# Autodesk Inventor assembly: Robot_Klara
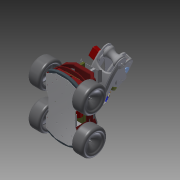
[picture p0: Inventor's stored thumbnail of the model, 180x180]
Saved by Autodesk Inventor 2015 (Build 190159000, 159)
## iProperties
Created: 2015-01-01
Part Number: Robot_Klara
Document SubType Name: Assembly
Designer: Turboslimak
Author: Turboslimak
## Documents named in this file (75)
- C:\Users\Turboslimak\Documents\Inventor\Robot_Klara\Robot_Klara.iam
- C:\Users\Turboslimak\Documents\Inventor\Robot_Klara\podvozek.ipt
- C:\Users\Turboslimak\Documents\Inventor\Robot_Klara\bocnice_kratsi.ipt
- C:\Users\Turboslimak\Documents\Inventor\Robot_Klara\kratka_prepazka.ipt
- C:\Users\Turboslimak\Documents\Inventor\Robot_Klara\predni_komatex.ipt
- C:\Users\Turboslimak\Documents\Inventor\Robot_Klara\bocnice_delsi.ipt
- C:\Users\Turboslimak\Documents\Inventor\Robot_Klara\prepazka_2x_lozisko_2x_dira.ipt
- C:\Users\Turboslimak\Documents\Inventor\Robot_Klara\hridel_kolo.ipt
- C:\Users\Turboslimak\Documents\Inventor\Robot_Klara\Lozisko_15mm.ipt
- C:\Users\Turboslimak\Documents\Inventor\Robot_Klara\hlavni_hridel.ipt
- C:\Users\Turboslimak\Documents\Inventor\Robot_Klara\prepazka_2x_lozisko_2x_dira_predni.ipt
- C:\Users\Turboslimak\Documents\Inventor\Robot_Klara\prepazka_2x_lozisko_1x_dira.ipt
- C:\Users\Turboslimak\Documents\Inventor\Robot_Klara\drzak_motory.ipt
- C:\Users\Turboslimak\Documents\Inventor\Robot_Klara\DC_motor+enkoder.ipt
- C:\Users\Turboslimak\Documents\Inventor\Robot_Klara\gear hridel.ipt
- C:\Users\Turboslimak\Documents\Inventor\Robot_Klara\gear motor.ipt
- C:\Users\Turboslimak\Documents\Inventor\Robot_Klara\Robot_Klara\Design Accelerator\Spur Gears2.iam
- C:\Users\Turboslimak\Documents\Inventor\Robot_Klara\Robot_Klara\Design Accelerator\Spur Gears3.iam
- C:\Users\Turboslimak\Documents\Inventor\Robot_Klara\vymezovaci_trubicka.ipt
- C:\Users\Turboslimak\Documents\Inventor\Robot_Klara\hridel kuzelova kolecka.ipt
- C:\Users\Turboslimak\Documents\Inventor\Robot_Klara\Robot_Klara\Design Accelerator\Bevel Gears2.iam
- C:\Users\Turboslimak\Documents\Inventor\Robot_Klara\Robot_Klara\Design Accelerator\Bevel Gears3.iam
- C:\Users\Turboslimak\Documents\Inventor\Robot_Klara\Robot_Klara\Design Accelerator\Bevel Gears4.iam
- C:\Users\Turboslimak\Documents\Inventor\Robot_Klara\Robot_Klara\Design Accelerator\Bevel Gears7.iam
- C:\Users\Turboslimak\Documents\Inventor\Robot_Klara\naraznik_kryt.ipt
- C:\Users\Turboslimak\Documents\Inventor\Robot_Klara\naraznik.ipt
- C:\Users\Turboslimak\Documents\Inventor\Robot_Klara\kolo.ipt
- C:\Users\Turboslimak\Documents\Inventor\Robot_Klara\izolovaci_deska.ipt
- C:\Users\Turboslimak\Documents\Inventor\Robot_Klara\vrch.ipt
- C:\Users\Turboslimak\Documents\Inventor\Robot_Klara\drzak_svetlomet0.ipt
- C:\Users\Turboslimak\Documents\Inventor\Robot_Klara\svetlo_trubicka.ipt
- C:\Users\Turboslimak\Documents\Inventor\Robot_Klara\svetlo_mlecne_plexi.ipt
- C:\Users\Turboslimak\Documents\Inventor\Robot_Klara\komatex_senzor.ipt
- C:\Users\Turboslimak\Documents\Inventor\Robot_Klara\podpera_rameno.ipt
- C:\Users\Turboslimak\Documents\Inventor\Robot_Klara\podpera_deska_rameno.ipt
- C:\Users\Turboslimak\Documents\Inventor\Robot_Klara\deska-pod_otocny kruh.ipt
- C:\Users\Turboslimak\Documents\Inventor\Robot_Klara\podvozek_priklopny_kryt.ipt
- C:\Users\Turboslimak\Documents\Inventor\Robot_Klara\valecky_na_otocny_kruh.ipt
- C:\Users\Turboslimak\Documents\Inventor\Robot_Klara\otocni_kruh(svrchni).ipt
- C:\Users\Turboslimak\Documents\Inventor\Robot_Klara\hridelka1.ipt
- C:\Users\Turboslimak\Documents\Inventor\Robot_Klara\standart_servo.ipt
- C:\Users\Turboslimak\Documents\Inventor\Robot_Klara\servo_paka_dolu.ipt
- C:\Users\Turboslimak\Documents\Inventor\Robot_Klara\stojan2.ipt
- C:\Users\Turboslimak\Documents\Inventor\Robot_Klara\stojan2a.ipt
- C:\Users\Turboslimak\Documents\Inventor\Robot_Klara\servodrzak.ipt
- C:\Users\Turboslimak\Documents\Inventor\Robot_Klara\micro_servo.ipt
- C:\Users\Turboslimak\Documents\Inventor\Robot_Klara\rameno(b)dole.ipt
- C:\Users\Turboslimak\Documents\Inventor\Robot_Klara\rameno(a)dole.ipt
- C:\Users\Turboslimak\Documents\Inventor\Robot_Klara\vystuha_hridel_nahore.ipt
- C:\Users\Turboslimak\Documents\Inventor\Robot_Klara\rameno(a)nahore.ipt
- C:\Users\Turboslimak\Documents\Inventor\Robot_Klara\rameno(b)nahore.ipt
- C:\Users\Turboslimak\Documents\Inventor\Robot_Klara\kolecko_servo(2).ipt
- C:\Users\Turboslimak\Documents\Inventor\Robot_Klara\kolecko_rameno(2).ipt
- C:\Users\Turboslimak\Documents\Inventor\Robot_Klara\clanek3a.ipt
- C:\Users\Turboslimak\Documents\Inventor\Robot_Klara\packa_strana(a).ipt
- C:\Users\Turboslimak\Documents\Inventor\Robot_Klara\otaceni_packy_microservo.ipt
- C:\Users\Turboslimak\Documents\Inventor\Robot_Klara\kolecko_rameno(3).ipt
- C:\Users\Turboslimak\Documents\Inventor\Robot_Klara\kolecko_servo(3).ipt
- C:\Users\Turboslimak\Documents\Inventor\Robot_Klara\hridel1.ipt
- C:\Users\Turboslimak\Documents\Inventor\Robot_Klara\hridel2.ipt
- C:\Users\Turboslimak\Documents\Inventor\Robot_Klara\hridelka_packa.ipt
- C:\Users\Turboslimak\Documents\Inventor\Robot_Klara\ruka_zak, deska.ipt
- C:\Users\Turboslimak\Documents\Inventor\Robot_Klara\tahlo3.ipt
- C:\Users\Turboslimak\Documents\Inventor\Robot_Klara\tahlo6.ipt
- C:\Users\Turboslimak\Documents\Inventor\Robot_Klara\tahlo7.ipt
- C:\Users\Turboslimak\Documents\Inventor\Robot_Klara\tahlo-neco.ipt
- C:\Users\Turboslimak\Documents\Inventor\Robot_Klara\tahlo5.ipt
- C:\Users\Turboslimak\Documents\Inventor\Robot_Klara\ruka_lozisko.ipt
- C:\Users\Turboslimak\Documents\Inventor\Robot_Klara\kolejnicka_ruka.ipt
- C:\Users\Turboslimak\Documents\Inventor\Robot_Klara\kolejnicka_ruka_druha_cast.ipt
- C:\Users\Turboslimak\Documents\Inventor\Robot_Klara\paka2_micro.ipt
- C:\Users\Turboslimak\Documents\Inventor\Robot_Klara\pracka_leva1.ipt
- C:\Users\Turboslimak\Documents\Inventor\Robot_Klara\packa_prava.ipt
- C:\Users\Turboslimak\Documents\Inventor\Robot_Klara\ruka_tahlo.ipt
- C:\Users\Turboslimak\Documents\Inventor\Robot_Klara\paka_packa.ipt
## Components (133 placed, 70 different names)
1. podvozek:1 — Mate:1, Mate:2, Mate:3, Mate:4, Mate:5, Mate:6, Mate:18, Mate:19, Mate:20, Mate:21, Mate:22, Mate:23, Mate:33, Mate:34, Mate:35, Mate:36, Mate:40, Mate:42, Mate:50, Flush:1, Mate:69, Mate:79, Mate:80, Mate:81, Mate:82, Mate:83, Mate:84, Mate:85, Mate:86, Mate:99, Mate:100, Mate:101, Mate:105, Mate:112, Mate:113, Mate:114, Mate:115, Mate:177, Mate:178, Mate:179, Mate:180, Mate:187, Mate:188, Mate:189, Mate:191, Mate:192, Mate:193, Mate:203, Mate:204, Mate:205
2. bocnice_kratsi:1 — Mate:4, Mate:5, Mate:6, Mate:24, Mate:74, Mate:75, Mate:225
3. bocnice_kratsi:2 — Mate:1, Mate:2, Mate:3, Mate:46, Mate:65, Mate:76, Mate:223
4. bocnice_delsi:1 — Mate:18, Mate:19, Mate:20, Mate:21, Mate:51, Mate:58, Mate:73
5. predni_komatex:1 — Mate:22, Mate:23, Mate:24, Mate:87, Mate:88, Mate:212, Mate:213, Mate:214, Mate:215, Mate:216, Mate:217
6. bocnice_delsi:2 — Mate:33, Mate:34, Mate:35, Mate:36, Mate:59, Mate:67
7. prepazka_2x_lozisko_2x_dira:1 — Mate:40, Mate:42, Mate:56, Mate:57, Mate:69, Mate:70, Mate:71, Mate:72, Mate:89, Mate:90, Flush:2, Flush:3
8. hridel_kolo:2 — Mate:51, Mate:139, Mate:146, Flush:9, Mate:164
9. hridel_kolo:4 — Mate:46, Mate:138, Mate:150, Flush:4
10. Lozisko_15mm:1 — Mate:57, Mate:102
11. Lozisko_15mm:2 — Mate:70, Mate:71, Mate:78
12. Lozisko_15mm:4 — Mate:222
13. Lozisko_15mm:5 — Mate:56, Mate:72, Mate:77
14. Lozisko_15mm:6 — Mate:58, Mate:73, Mate:142
15. Lozisko_15mm:8 — Mate:65, Mate:76, Mate:143
16. Lozisko_15mm:10 — Mate:59, Mate:67, Mate:145
17. kratka_prepazka:1 — Mate:79, Mate:80, Mate:90, Mate:91, Mate:92, Mate:129
18. kratka_prepazka:2 — Mate:82, Mate:84, Mate:89, Mate:93, Mate:94
19. kratka_prepazka:3 — Mate:83, Mate:85, Mate:88, Mate:95, Mate:98
20. kratka_prepazka:4 — Mate:81, Mate:86, Mate:87, Mate:96, Mate:97, Mate:239
21. hlavni_hridel:1 — Mate:78, Mate:111, Flush:3, Mate:123, Mate:152, Flush:6, Mate:154, Mate:160, Mate:167
22. hlavni_hridel:2 — Mate:77, Mate:103, Mate:110, Flush:2, Mate:122, Mate:147, Mate:153, Flush:5, Mate:157, Mate:163
23. Lozisko_15mm:11 — Mate:93, Mate:94
24. Lozisko_15mm:12 — Mate:91, Mate:92, Mate:175
25. Lozisko_15mm:13 — Mate:95, Mate:98
26. Lozisko_15mm:14 — Mate:74, Mate:75, Mate:144
27. Lozisko_15mm:15 — Mate:96, Mate:97, Mate:173
28. prepazka_2x_lozisko_2x_dira_predni:1 — Mate:99, Mate:100, Mate:101, Mate:102, Mate:104
29. Lozisko_15mm:16 — Mate:106, Mate:109, Mate:111
30. Lozisko_15mm:17 — Mate:107, Mate:108, Mate:110
31. Lozisko_15mm:18 — Mate:103, Mate:104
32. prepazka_2x_lozisko_1x_dira:1 — Mate:105, Mate:106, Mate:107, Mate:108, Mate:109, Mate:112, Mate:126, Mate:127, Mate:128, Mate:224
33. drzak_motory:1 — Mate:113, Mate:114, Mate:115, Mate:116, Mate:117, Mate:118, Mate:119, Mate:120, Mate:121
34. DC_motor+enkoder:1 — Mate:117, Mate:119, Mate:120, Mate:125
35. DC_motor+enkoder:2 — Mate:116, Mate:118, Mate:121, Mate:124
36. gear hridel:1 — Mate:122, Mate:126, Mate:132, Mate:133
37. gear hridel:2 — Mate:123, Mate:127, Mate:136, Mate:137
38. gear motor:1 — Mate:125, Mate:129, Mate:134, Mate:135
39. gear motor:2 — Mate:124, Mate:128, Mate:130, Mate:131
40. Spur Gears:1 [sub-assembly] — Mate:130, Mate:131, Mate:132, Mate:133
41. Spur Gears:2 [sub-assembly] — Mate:134, Mate:135, Mate:136, Mate:137
42. vymezovaci_trubicka:1 — Mate:138, Mate:143, Mate:195, Mate:196
43. vymezovaci_trubicka:2 — Mate:139, Mate:142, Mate:197, Mate:198
44. vymezovaci_trubicka:3 — Mate:144, Mate:172, Mate:201, Mate:202
45. vymezovaci_trubicka:4 — Mate:145, Mate:176, Mate:199
46. hridel kuzelova kolecka:1 — Mate:150, Flush:4, Mate:157, Mate:162, Angle:3
47. hridel kuzelova kolecka:2 — Mate:154, Angle:1, Mate:159, Flush:10
48. hridel kuzelova kolecka:3 — Mate:152, Flush:6, Mate:158
49. hridel kuzelova kolecka:4 — Mate:153, Flush:5, Mate:161, Angle:2
50. hridel kuzelova kolecka:5 — Mate:167, Mate:169, Mate:170
51. hridel kuzelova kolecka:6 — Mate:168, Angle:4, Mate:171, Flush:11, Mate:221
52. hridel kuzelova kolecka:7 — Mate:146, Flush:9, Mate:165
53. hridel kuzelova kolecka:8 — Mate:147, Mate:166
54. Bevel Gears:1 [sub-assembly] — Angle:1, Mate:158, Mate:159, Mate:160, Mate:174
55. Bevel Gears:2 [sub-assembly] — Mate:161, Angle:2, Mate:162, Angle:3
56. Bevel Gears:3 [sub-assembly] — Mate:163, Mate:164, Mate:165, Mate:166
57. Bevel Gears:4 [sub-assembly] — Mate:168, Angle:4, Mate:169, Mate:170, Mate:171
58. hridel_kolo:5 — Flush:11, Mate:175, Mate:176, Mate:200, Mate:221, Mate:222
59. hridel_kolo:6 — Flush:10, Mate:172, Mate:173, Mate:174
60. naraznik_kryt:1 — Mate:177, Mate:178, Mate:190
61. naraznik_kryt:2 — Mate:179, Mate:180, Mate:194
62. naraznik:2 — Mate:187, Mate:188, Mate:189, Mate:190
63. naraznik:3 — Mate:191, Mate:192, Mate:193, Mate:194
64. kolo:1 — Mate:199, Mate:200
65. kolo:2 — Mate:197, Mate:198
66. kolo:3 — Mate:201, Mate:202
67. kolo:4 — Mate:195, Mate:196
68. izolovaci_deska:1 — Mate:203, Mate:204, Mate:205
69. vrch:1 — Mate:223, Mate:224, Mate:225, Mate:226, Flush:12, Mate:228, Mate:229, Mate:230, Mate:231, Mate:236, Mate:237, Mate:238, Mate:241, Mate:242, Mate:243, Mate:244
70. drzak_svetlomet0:1 — Mate:212, Mate:213, Mate:214, Mate:215, Mate:216, Mate:218
71. svetlo_trubicka:1 — Mate:217, Mate:218, Mate:219, Mate:220
72. svetlo_mlecne_plexi:1 — Mate:219, Mate:220
73. komatex_senzor:1 — Mate:226, Flush:12
74. podpera_rameno:1 — Mate:228, Mate:229, Mate:235
75. podpera_rameno:2 — Mate:230, Mate:231, Mate:232, Mate:234
76. podpera_deska_rameno:1 — Mate:232, Mate:234, Mate:235
77. deska-pod_otocny kruh:1 — Mate:236, Mate:237, Mate:238
78. podvozek_priklopny_kryt:1 — Mate:239, Mate:241
79. deska-pod_otocny kruh:2 — Mate:242, Mate:243, Mate:244, Mate:245, Mate:246, Mate:247, Mate:248, Mate:249, Mate:250, Mate:251
80. valecky_na_otocny_kruh:1 — Mate:245, Mate:246, Tangent:1
81. valecky_na_otocny_kruh:2 — Mate:249, Mate:250, Tangent:2
82. valecky_na_otocny_kruh:3 — Mate:247, Mate:248
83. otocni_kruh(svrchni):1 — Tangent:1, Tangent:2, Mate:252, Mate:253, Mate:254, Mate:255, Mate:264, Mate:265, Mate:266, Mate:267, Mate:268, Mate:269, Mate:274
84. hridelka1:1 — Mate:251, Mate:252
85. standart_servo:1 — Mate:253, Mate:254, Mate:255, Mate:262, Mate:263
86. servo_paka_dolu:1 — Mate:262, Mate:263, Mate:275, Mate:276, Mate:277
87. stojan2:1 — Mate:264, Mate:265, Mate:270, Mate:274, Mate:282, Mate:318
88. stojan2a:1 — Mate:266, Mate:267, Mate:268
89. servodrzak:1 — Mate:269, Mate:270, Mate:271, Mate:272, Mate:273
90. micro_servo:1 — Mate:271, Mate:272, Mate:273
91. rameno(b)dole:1 — Mate:275, Mate:276, Mate:277, Mate:278, Mate:279, Mate:280, Mate:281, Mate:283, Mate:295
92. standart_servo:2 — Mate:278, Mate:279, Mate:280, Mate:290, Mate:291
93. rameno(a)dole:1 — Mate:281, Mate:282, Mate:283, Mate:289, Mate:316
94. vystuha_hridel_nahore:1 — Mate:284, Mate:285, Mate:286, Mate:287, Mate:289
95. rameno(a)nahore:1 — Mate:284, Mate:285, Mate:288, Mate:308, Mate:309, Mate:310, Mate:313, Mate:317
96. rameno(b)nahore:1 — Mate:286, Mate:287, Mate:288, Mate:292, Mate:293, Mate:294, Mate:312
97. kolecko_servo(2):1 — Mate:290, Mate:291
98. kolecko_rameno(2):1 — Mate:292, Mate:293, Mate:294, Mate:295
99. standart_servo:3 — Mate:296, Mate:297, Mate:298, Mate:306, Mate:307
100. clanek3a:1 — Mate:299, Mate:300, Mate:301, Mate:304, Mate:305, Mate:311, Mate:312, Mate:380
101. packa_strana(a):1 — Mate:296, Mate:297, Mate:298, Mate:304, Mate:305, Mate:311
102. micro_servo:2 — Mate:299, Mate:300, Mate:301, Mate:302, Mate:303
103. otaceni_packy_microservo:1 — Mate:302, Mate:303, Mate:314, Mate:315
104. kolecko_rameno(3):1 — Mate:308, Mate:309, Mate:310
105. kolecko_servo(3):1 — Mate:306, Mate:307, Mate:313
106. hridel1:1 — Mate:316
107. hridel2:1 — Mate:317
108. hridelka_packa:1 — Mate:314, Mate:315, Mate:373
109. hridel1:2 — Mate:318
110. ruka_zak, deska:1 — Mate:319, Mate:320, Mate:326, Mate:328, Mate:330, Mate:331, Mate:332, Mate:333, Mate:334, Mate:336, Mate:343, Mate:344, Mate:346, Mate:347, Mate:349, Mate:350, Mate:351, Mate:352, Mate:353, Mate:354, Mate:362, Mate:363, Mate:364, Mate:366, Mate:377, Mate:378, Mate:392, Mate:393, Mate:394
111. tahlo3:1 — Mate:319, Mate:320, Mate:368, Mate:395
112. tahlo7:1 — Mate:366, Mate:370, Mate:372
113. tahlo-neco:1 — Mate:368, Mate:369, Mate:370, Mate:388
114. ruka_lozisko:1 — Mate:362, Mate:363, Mate:364, Mate:373, Mate:380
115. kolejnicka_ruka:1 — Mate:349, Mate:350, Mate:351, Mate:357, Mate:358
116. kolejnicka_ruka_druha_cast:1 — Mate:357, Mate:358, Mate:384, Mate:385, Mate:386
117. paka2_micro:1 — Mate:355, Mate:356, Mate:374, Mate:389
118. pracka_leva1:1 — Mate:327, Mate:329, Mate:335, Mate:348, Mate:395
119. ruka_tahlo:1 — Mate:326, Mate:327, Mate:328, Mate:329
120. ruka_tahlo:2 — Mate:332, Mate:336, Mate:337
121. ruka_tahlo:3 — Mate:333, Mate:334, Mate:335
122. ruka_tahlo:4 — Mate:330, Mate:331, Mate:337, Mate:383
123. tahlo3:2 — Mate:343, Mate:344, Mate:375, Mate:376
124. tahlo3:3 — Mate:346, Mate:347, Mate:348, Mate:369
125. tahlo3:4 — Mate:377, Mate:378, Mate:379, Mate:381, Mate:382
126. micro_servo:3 — Mate:352, Mate:353, Mate:354, Mate:355, Mate:356
127. tahlo-neco:2
128. tahlo-neco:3 — Mate:372, Mate:375, Mate:376, Mate:379, Mate:387
129. tahlo5:1 — Mate:374
130. packa_prava:1 — Mate:381, Mate:382, Mate:383
131. tahlo6:1 — Mate:384, Mate:385, Mate:386, Mate:387, Mate:388, Mate:390, Mate:391
132. tahlo5:2 — Mate:389, Mate:390, Mate:391
133. paka_packa:1 — Mate:392, Mate:393, Mate:394
## Relationships (326: Mate 310, Flush 10, Angle 4, Tangent 2)
- Mate:1: podvozek:1 ↔ bocnice_kratsi:2
- Mate:2: podvozek:1 ↔ bocnice_kratsi:2
- Mate:3: podvozek:1 ↔ bocnice_kratsi:2
- Mate:4: podvozek:1 ↔ bocnice_kratsi:1
- Mate:5: podvozek:1 ↔ bocnice_kratsi:1
- Mate:6: podvozek:1 ↔ bocnice_kratsi:1
- Mate:18: podvozek:1 ↔ bocnice_delsi:1
- Mate:19: podvozek:1 ↔ bocnice_delsi:1
- Mate:20: podvozek:1 ↔ bocnice_delsi:1
- Mate:21: podvozek:1 ↔ bocnice_delsi:1
- Mate:22: podvozek:1 ↔ predni_komatex:1
- Mate:23: podvozek:1 ↔ predni_komatex:1
- Mate:24: bocnice_kratsi:1 ↔ predni_komatex:1
- Mate:33: podvozek:1 ↔ bocnice_delsi:2
- Mate:34: podvozek:1 ↔ bocnice_delsi:2
- Mate:35: podvozek:1 ↔ bocnice_delsi:2
- Mate:36: podvozek:1 ↔ bocnice_delsi:2
- Mate:40: podvozek:1 ↔ prepazka_2x_lozisko_2x_dira:1
- Mate:42: podvozek:1 ↔ prepazka_2x_lozisko_2x_dira:1
- Mate:46: bocnice_kratsi:2 ↔ hridel_kolo:4
- Mate:50: podvozek:1
- Flush:1: podvozek:1
- Mate:51: bocnice_delsi:1 ↔ hridel_kolo:2
- Mate:56: prepazka_2x_lozisko_2x_dira:1 ↔ Lozisko_15mm:5
- Mate:57: prepazka_2x_lozisko_2x_dira:1 ↔ Lozisko_15mm:1
- Mate:58: bocnice_delsi:1 ↔ Lozisko_15mm:6
- Mate:59: bocnice_delsi:2 ↔ Lozisko_15mm:10
- Mate:65: bocnice_kratsi:2 ↔ Lozisko_15mm:8
- Mate:67: bocnice_delsi:2 ↔ Lozisko_15mm:10
- Mate:69: podvozek:1 ↔ prepazka_2x_lozisko_2x_dira:1
- Mate:70: prepazka_2x_lozisko_2x_dira:1 ↔ Lozisko_15mm:2
- Mate:71: prepazka_2x_lozisko_2x_dira:1 ↔ Lozisko_15mm:2
- Mate:72: prepazka_2x_lozisko_2x_dira:1 ↔ Lozisko_15mm:5
- Mate:73: bocnice_delsi:1 ↔ Lozisko_15mm:6
- Mate:74: bocnice_kratsi:1 ↔ Lozisko_15mm:14
- Mate:75: bocnice_kratsi:1 ↔ Lozisko_15mm:14
- Mate:76: bocnice_kratsi:2 ↔ Lozisko_15mm:8
- Mate:77: Lozisko_15mm:5 ↔ hlavni_hridel:2
- Mate:78: Lozisko_15mm:2 ↔ hlavni_hridel:1
- Mate:79: podvozek:1 ↔ kratka_prepazka:1
- Mate:80: podvozek:1 ↔ kratka_prepazka:1
- Mate:81: podvozek:1 ↔ kratka_prepazka:4
- Mate:82: podvozek:1 ↔ kratka_prepazka:2
- Mate:83: podvozek:1 ↔ kratka_prepazka:3
- Mate:84: podvozek:1 ↔ kratka_prepazka:2
- Mate:85: podvozek:1 ↔ kratka_prepazka:3
- Mate:86: podvozek:1 ↔ kratka_prepazka:4
- Mate:87: predni_komatex:1 ↔ kratka_prepazka:4
- Mate:88: predni_komatex:1 ↔ kratka_prepazka:3
- Mate:89: prepazka_2x_lozisko_2x_dira:1 ↔ kratka_prepazka:2
- Mate:90: prepazka_2x_lozisko_2x_dira:1 ↔ kratka_prepazka:1
- Mate:91: kratka_prepazka:1 ↔ Lozisko_15mm:12
- Mate:92: kratka_prepazka:1 ↔ Lozisko_15mm:12
- Mate:93: kratka_prepazka:2 ↔ Lozisko_15mm:11
- Mate:94: kratka_prepazka:2 ↔ Lozisko_15mm:11
- Mate:95: kratka_prepazka:3 ↔ Lozisko_15mm:13
- Mate:96: kratka_prepazka:4 ↔ Lozisko_15mm:15
- Mate:97: kratka_prepazka:4 ↔ Lozisko_15mm:15
- Mate:98: kratka_prepazka:3 ↔ Lozisko_15mm:13
- Mate:99: podvozek:1 ↔ prepazka_2x_lozisko_2x_dira_predni:1
- Mate:100: podvozek:1 ↔ prepazka_2x_lozisko_2x_dira_predni:1
- Mate:101: podvozek:1 ↔ prepazka_2x_lozisko_2x_dira_predni:1
- Mate:102: Lozisko_15mm:1 ↔ prepazka_2x_lozisko_2x_dira_predni:1
- Mate:103: hlavni_hridel:2 ↔ Lozisko_15mm:18
- Mate:104: prepazka_2x_lozisko_2x_dira_predni:1 ↔ Lozisko_15mm:18
- Mate:105: podvozek:1 ↔ prepazka_2x_lozisko_1x_dira:1
- Mate:106: Lozisko_15mm:16 ↔ prepazka_2x_lozisko_1x_dira:1
- Mate:107: Lozisko_15mm:17 ↔ prepazka_2x_lozisko_1x_dira:1
- Mate:108: Lozisko_15mm:17 ↔ prepazka_2x_lozisko_1x_dira:1
- Mate:109: Lozisko_15mm:16 ↔ prepazka_2x_lozisko_1x_dira:1
- Mate:110: hlavni_hridel:2 ↔ Lozisko_15mm:17
- Mate:111: hlavni_hridel:1 ↔ Lozisko_15mm:16
- Mate:112: podvozek:1 ↔ prepazka_2x_lozisko_1x_dira:1
- Mate:113: podvozek:1 ↔ drzak_motory:1
- Mate:114: podvozek:1 ↔ drzak_motory:1
- Mate:115: podvozek:1 ↔ drzak_motory:1
- Flush:2: prepazka_2x_lozisko_2x_dira:1 ↔ hlavni_hridel:2
- Flush:3: prepazka_2x_lozisko_2x_dira:1 ↔ hlavni_hridel:1
- Mate:116: drzak_motory:1 ↔ DC_motor+enkoder:2
- Mate:117: drzak_motory:1 ↔ DC_motor+enkoder:1
- Mate:118: drzak_motory:1 ↔ DC_motor+enkoder:2
- Mate:119: drzak_motory:1 ↔ DC_motor+enkoder:1
- Mate:120: drzak_motory:1 ↔ DC_motor+enkoder:1
- Mate:121: drzak_motory:1 ↔ DC_motor+enkoder:2
- Mate:122: hlavni_hridel:2 ↔ gear hridel:1
- Mate:123: hlavni_hridel:1 ↔ gear hridel:2
- Mate:124: DC_motor+enkoder:2 ↔ gear motor:2
- Mate:125: DC_motor+enkoder:1 ↔ gear motor:1
- Mate:126 (3 mm): prepazka_2x_lozisko_1x_dira:1 ↔ gear hridel:1
- Mate:127 (3 mm): prepazka_2x_lozisko_1x_dira:1 ↔ gear hridel:2
- Mate:128 (3 mm): prepazka_2x_lozisko_1x_dira:1 ↔ gear motor:2
- Mate:129 (3 mm): kratka_prepazka:1 ↔ gear motor:1
- Mate:130: gear motor:2 ↔ Spur Gears:1
- Mate:131: gear motor:2 ↔ Spur Gears:1
- Mate:132: gear hridel:1 ↔ Spur Gears:1
- Mate:133: gear hridel:1 ↔ Spur Gears:1
- Mate:134: gear motor:1 ↔ Spur Gears:2
- Mate:135: gear motor:1 ↔ Spur Gears:2
- Mate:136: gear hridel:2 ↔ Spur Gears:2
- Mate:137: gear hridel:2 ↔ Spur Gears:2
- Mate:138: hridel_kolo:4 ↔ vymezovaci_trubicka:1
- Mate:139: hridel_kolo:2 ↔ vymezovaci_trubicka:2
- Mate:142: Lozisko_15mm:6 ↔ vymezovaci_trubicka:2
- Mate:143: Lozisko_15mm:8 ↔ vymezovaci_trubicka:1
- Mate:144: Lozisko_15mm:14 ↔ vymezovaci_trubicka:3
- Mate:145: Lozisko_15mm:10 ↔ vymezovaci_trubicka:4
- Mate:146: hridel_kolo:2 ↔ hridel kuzelova kolecka:7
- Mate:147: hlavni_hridel:2 ↔ hridel kuzelova kolecka:8
- Mate:150: hridel_kolo:4 ↔ hridel kuzelova kolecka:1
- Mate:152: hlavni_hridel:1 ↔ hridel kuzelova kolecka:3
- Mate:153: hlavni_hridel:2 ↔ hridel kuzelova kolecka:4
- Flush:4: hridel_kolo:4 ↔ hridel kuzelova kolecka:1
- Flush:5: hlavni_hridel:2 ↔ hridel kuzelova kolecka:4
- Flush:6: hlavni_hridel:1 ↔ hridel kuzelova kolecka:3
- Flush:9: hridel_kolo:2 ↔ hridel kuzelova kolecka:7
- Mate:154 (4.8 mm): hlavni_hridel:1 ↔ hridel kuzelova kolecka:2
- Mate:157 (4.8 mm): hlavni_hridel:2 ↔ hridel kuzelova kolecka:1
- Angle:1 (0 deg): hridel kuzelova kolecka:2 ↔ Bevel Gears:1
- Mate:158: hridel kuzelova kolecka:3 ↔ Bevel Gears:1
- Mate:159: hridel kuzelova kolecka:2 ↔ Bevel Gears:1
- Mate:160: hlavni_hridel:1 ↔ Bevel Gears:1
- Mate:161: hridel kuzelova kolecka:4 ↔ Bevel Gears:2
- Angle:2 (0 deg): hridel kuzelova kolecka:4 ↔ Bevel Gears:2
- Mate:162: hridel kuzelova kolecka:1 ↔ Bevel Gears:2
- Angle:3 (0 deg): hridel kuzelova kolecka:1 ↔ Bevel Gears:2
- Mate:163: hlavni_hridel:2 ↔ Bevel Gears:3
- Mate:164: hridel_kolo:2 ↔ Bevel Gears:3
- Mate:165: hridel kuzelova kolecka:7 ↔ Bevel Gears:3
- Mate:166: hridel kuzelova kolecka:8 ↔ Bevel Gears:3
- Mate:167: hlavni_hridel:1 ↔ hridel kuzelova kolecka:5
- Mate:168: hridel kuzelova kolecka:6 ↔ Bevel Gears:4
- Angle:4 (0 deg): hridel kuzelova kolecka:6 ↔ Bevel Gears:4
- Mate:169: hridel kuzelova kolecka:5 ↔ Bevel Gears:4
- Mate:170: hridel kuzelova kolecka:5 ↔ Bevel Gears:4
- Mate:171: hridel kuzelova kolecka:6 ↔ Bevel Gears:4
- Flush:10: hridel kuzelova kolecka:2 ↔ hridel_kolo:6
- Mate:172: vymezovaci_trubicka:3 ↔ hridel_kolo:6
- Mate:173: Lozisko_15mm:15 ↔ hridel_kolo:6
- Mate:174: Bevel Gears:1 ↔ hridel_kolo:6
- Flush:11: hridel kuzelova kolecka:6 ↔ hridel_kolo:5
- Mate:175: Lozisko_15mm:12 ↔ hridel_kolo:5
- Mate:176: vymezovaci_trubicka:4 ↔ hridel_kolo:5
- Mate:177: podvozek:1 ↔ naraznik_kryt:1
- Mate:178: podvozek:1 ↔ naraznik_kryt:1
- Mate:179: podvozek:1 ↔ naraznik_kryt:2
- Mate:180: podvozek:1 ↔ naraznik_kryt:2
- Mate:187: podvozek:1 ↔ naraznik:2
- Mate:188: podvozek:1 ↔ naraznik:2
- Mate:189: podvozek:1 ↔ naraznik:2
- Mate:190: naraznik_kryt:1 ↔ naraznik:2
- Mate:191: podvozek:1 ↔ naraznik:3
- Mate:192: podvozek:1 ↔ naraznik:3
- Mate:193: podvozek:1 ↔ naraznik:3
- Mate:194: naraznik_kryt:2 ↔ naraznik:3
- Mate:195: vymezovaci_trubicka:1 ↔ kolo:4
- Mate:196: vymezovaci_trubicka:1 ↔ kolo:4
- Mate:197: vymezovaci_trubicka:2 ↔ kolo:2
- Mate:198: vymezovaci_trubicka:2 ↔ kolo:2
- Mate:199: vymezovaci_trubicka:4 ↔ kolo:1
- Mate:200: hridel_kolo:5 ↔ kolo:1
- Mate:201: vymezovaci_trubicka:3 ↔ kolo:3
- Mate:202: vymezovaci_trubicka:3 ↔ kolo:3
- Mate:203: podvozek:1 ↔ izolovaci_deska:1
- Mate:204: podvozek:1 ↔ izolovaci_deska:1
- Mate:205: podvozek:1 ↔ izolovaci_deska:1
- Mate:212: predni_komatex:1 ↔ drzak_svetlomet0:1
- Mate:213: predni_komatex:1 ↔ drzak_svetlomet0:1
- Mate:214: predni_komatex:1 ↔ drzak_svetlomet0:1
- Mate:215: predni_komatex:1 ↔ drzak_svetlomet0:1
- Mate:216: predni_komatex:1 ↔ drzak_svetlomet0:1
- Mate:217: predni_komatex:1 ↔ svetlo_trubicka:1
- Mate:218: drzak_svetlomet0:1 ↔ svetlo_trubicka:1
- Mate:219: svetlo_trubicka:1 ↔ svetlo_mlecne_plexi:1
- Mate:220: svetlo_trubicka:1 ↔ svetlo_mlecne_plexi:1
- Mate:221: hridel kuzelova kolecka:6 ↔ hridel_kolo:5
- Mate:222: Lozisko_15mm:4 ↔ hridel_kolo:5
- Mate:223: bocnice_kratsi:2 ↔ vrch:1
- Mate:224: prepazka_2x_lozisko_1x_dira:1 ↔ vrch:1
- Mate:225: bocnice_kratsi:1 ↔ vrch:1
- Mate:226: vrch:1 ↔ komatex_senzor:1
- Flush:12: vrch:1 ↔ komatex_senzor:1
- Mate:228: vrch:1 ↔ podpera_rameno:1
- Mate:229: vrch:1 ↔ podpera_rameno:1
- Mate:230: vrch:1 ↔ podpera_rameno:2
- Mate:231: vrch:1 ↔ podpera_rameno:2
- Mate:232: podpera_rameno:2 ↔ podpera_deska_rameno:1
- Mate:234: podpera_rameno:2 ↔ podpera_deska_rameno:1
- Mate:235: podpera_rameno:1 ↔ podpera_deska_rameno:1
- Mate:236: vrch:1 ↔ deska-pod_otocny kruh:1
- Mate:237: vrch:1 ↔ deska-pod_otocny kruh:1
- Mate:238: vrch:1 ↔ deska-pod_otocny kruh:1
- Mate:239: kratka_prepazka:4 ↔ podvozek_priklopny_kryt:1
- Mate:241 (3 mm): vrch:1 ↔ podvozek_priklopny_kryt:1
- Mate:242: vrch:1 ↔ deska-pod_otocny kruh:2
- Mate:243: vrch:1 ↔ deska-pod_otocny kruh:2
- Mate:244: vrch:1 ↔ deska-pod_otocny kruh:2
- Mate:245: deska-pod_otocny kruh:2 ↔ valecky_na_otocny_kruh:1
- Mate:246 (0.2 mm): deska-pod_otocny kruh:2 ↔ valecky_na_otocny_kruh:1
- Mate:247: deska-pod_otocny kruh:2 ↔ valecky_na_otocny_kruh:3
- Mate:248 (0.2 mm): deska-pod_otocny kruh:2 ↔ valecky_na_otocny_kruh:3
- Mate:249: deska-pod_otocny kruh:2 ↔ valecky_na_otocny_kruh:2
- Mate:250 (0.2 mm): deska-pod_otocny kruh:2 ↔ valecky_na_otocny_kruh:2
- Mate:251: deska-pod_otocny kruh:2 ↔ hridelka1:1
- Tangent:1: valecky_na_otocny_kruh:1 ↔ otocni_kruh(svrchni):1
- Tangent:2: valecky_na_otocny_kruh:2 ↔ otocni_kruh(svrchni):1
- Mate:252: otocni_kruh(svrchni):1 ↔ hridelka1:1
- Mate:253: otocni_kruh(svrchni):1 ↔ standart_servo:1
- Mate:254: otocni_kruh(svrchni):1 ↔ standart_servo:1
- Mate:255: otocni_kruh(svrchni):1 ↔ standart_servo:1
- Mate:262: standart_servo:1 ↔ servo_paka_dolu:1
- Mate:263 (0.5 mm): standart_servo:1 ↔ servo_paka_dolu:1
- Mate:264: otocni_kruh(svrchni):1 ↔ stojan2:1
- Mate:265: otocni_kruh(svrchni):1 ↔ stojan2:1
- Mate:266: otocni_kruh(svrchni):1 ↔ stojan2a:1
- Mate:267: otocni_kruh(svrchni):1 ↔ stojan2a:1
- Mate:268: otocni_kruh(svrchni):1 ↔ stojan2a:1
- Mate:269: otocni_kruh(svrchni):1 ↔ servodrzak:1
- Mate:270 (0.3 mm): stojan2:1 ↔ servodrzak:1
- Mate:271: servodrzak:1 ↔ micro_servo:1
- Mate:272: servodrzak:1 ↔ micro_servo:1
- Mate:273: servodrzak:1 ↔ micro_servo:1
- Mate:274: otocni_kruh(svrchni):1 ↔ stojan2:1
- Mate:275: servo_paka_dolu:1 ↔ rameno(b)dole:1
- Mate:276: servo_paka_dolu:1 ↔ rameno(b)dole:1
- Mate:277: servo_paka_dolu:1 ↔ rameno(b)dole:1
- Mate:278: rameno(b)dole:1 ↔ standart_servo:2
- Mate:279: rameno(b)dole:1 ↔ standart_servo:2
- Mate:280: rameno(b)dole:1 ↔ standart_servo:2
- Mate:281: rameno(b)dole:1 ↔ rameno(a)dole:1
- Mate:282: stojan2:1 ↔ rameno(a)dole:1
- Mate:283: rameno(b)dole:1 ↔ rameno(a)dole:1
- Mate:284: vystuha_hridel_nahore:1 ↔ rameno(a)nahore:1
- Mate:285: vystuha_hridel_nahore:1 ↔ rameno(a)nahore:1
- Mate:286: vystuha_hridel_nahore:1 ↔ rameno(b)nahore:1
- Mate:287: vystuha_hridel_nahore:1 ↔ rameno(b)nahore:1
- Mate:288: rameno(a)nahore:1 ↔ rameno(b)nahore:1
- Mate:289: rameno(a)dole:1 ↔ vystuha_hridel_nahore:1
- Mate:290 (0.4 mm): standart_servo:2 ↔ kolecko_servo(2):1
- Mate:291: standart_servo:2 ↔ kolecko_servo(2):1
- Mate:292: rameno(b)nahore:1 ↔ kolecko_rameno(2):1
- Mate:293: rameno(b)nahore:1 ↔ kolecko_rameno(2):1
- Mate:294 (2 mm): rameno(b)nahore:1 ↔ kolecko_rameno(2):1
- Mate:295 (2 mm): rameno(b)dole:1 ↔ kolecko_rameno(2):1
- Mate:296: standart_servo:3 ↔ packa_strana(a):1
- Mate:297: standart_servo:3 ↔ packa_strana(a):1
- Mate:298: standart_servo:3 ↔ packa_strana(a):1
- Mate:299: clanek3a:1 ↔ micro_servo:2
- Mate:300: clanek3a:1 ↔ micro_servo:2
- Mate:301: clanek3a:1 ↔ micro_servo:2
- Mate:302: micro_servo:2 ↔ otaceni_packy_microservo:1
- Mate:303: micro_servo:2 ↔ otaceni_packy_microservo:1
- Mate:304: clanek3a:1 ↔ packa_strana(a):1
- Mate:305: clanek3a:1 ↔ packa_strana(a):1
- Mate:306: standart_servo:3 ↔ kolecko_servo(3):1
- Mate:307: standart_servo:3 ↔ kolecko_servo(3):1
- Mate:308: rameno(a)nahore:1 ↔ kolecko_rameno(3):1
- Mate:309 (2 mm): rameno(a)nahore:1 ↔ kolecko_rameno(3):1
- Mate:310: rameno(a)nahore:1 ↔ kolecko_rameno(3):1
- Mate:311: clanek3a:1 ↔ packa_strana(a):1
- Mate:312: rameno(b)nahore:1 ↔ clanek3a:1
- Mate:313 (2 mm): rameno(a)nahore:1 ↔ kolecko_servo(3):1
- Mate:314: otaceni_packy_microservo:1 ↔ hridelka_packa:1
- Mate:315: otaceni_packy_microservo:1 ↔ hridelka_packa:1
- Mate:316: rameno(a)dole:1 ↔ hridel1:1
- Mate:317: rameno(a)nahore:1 ↔ hridel2:1
- Mate:318: stojan2:1 ↔ hridel1:2
- Mate:319: ruka_zak, deska:1 ↔ tahlo3:1
- Mate:320: ruka_zak, deska:1 ↔ tahlo3:1
- Mate:326: ruka_zak, deska:1 ↔ ruka_tahlo:1
- Mate:327: pracka_leva1:1 ↔ ruka_tahlo:1
- Mate:328: ruka_zak, deska:1 ↔ ruka_tahlo:1
- Mate:329: pracka_leva1:1 ↔ ruka_tahlo:1
- Mate:330: ruka_zak, deska:1 ↔ ruka_tahlo:4
- Mate:331: ruka_zak, deska:1 ↔ ruka_tahlo:4
- Mate:332: ruka_zak, deska:1 ↔ ruka_tahlo:2
- Mate:333: ruka_zak, deska:1 ↔ ruka_tahlo:3
- Mate:334: ruka_zak, deska:1 ↔ ruka_tahlo:3
- Mate:335: pracka_leva1:1 ↔ ruka_tahlo:3
- Mate:336: ruka_zak, deska:1 ↔ ruka_tahlo:2
- Mate:337: ruka_tahlo:2 ↔ ruka_tahlo:4
- Mate:343: ruka_zak, deska:1 ↔ tahlo3:2
- Mate:344: ruka_zak, deska:1 ↔ tahlo3:2
- Mate:346: ruka_zak, deska:1 ↔ tahlo3:3
- Mate:347: ruka_zak, deska:1 ↔ tahlo3:3
- Mate:348: pracka_leva1:1 ↔ tahlo3:3
- Mate:349: ruka_zak, deska:1 ↔ kolejnicka_ruka:1
- Mate:350: ruka_zak, deska:1 ↔ kolejnicka_ruka:1
- Mate:351: ruka_zak, deska:1 ↔ kolejnicka_ruka:1
- Mate:352: ruka_zak, deska:1 ↔ micro_servo:3
- Mate:353: ruka_zak, deska:1 ↔ micro_servo:3
- Mate:354: ruka_zak, deska:1 ↔ micro_servo:3
- Mate:355: paka2_micro:1 ↔ micro_servo:3
- Mate:356: paka2_micro:1 ↔ micro_servo:3
- Mate:357 (3 mm): kolejnicka_ruka:1 ↔ kolejnicka_ruka_druha_cast:1
- Mate:358 (4 mm): kolejnicka_ruka:1 ↔ kolejnicka_ruka_druha_cast:1
- Mate:362: ruka_zak, deska:1 ↔ ruka_lozisko:1
- Mate:363: ruka_zak, deska:1 ↔ ruka_lozisko:1
- Mate:364: ruka_zak, deska:1 ↔ ruka_lozisko:1
- Mate:366: ruka_zak, deska:1 ↔ tahlo7:1
- Mate:368: tahlo3:1 ↔ tahlo-neco:1
- Mate:369: tahlo-neco:1 ↔ tahlo3:3
- Mate:370: tahlo7:1 ↔ tahlo-neco:1
- Mate:372: tahlo7:1 ↔ tahlo-neco:3
- Mate:373: hridelka_packa:1 ↔ ruka_lozisko:1
- Mate:374: paka2_micro:1 ↔ tahlo5:1
- Mate:375: tahlo3:2 ↔ tahlo-neco:3
- Mate:376: tahlo3:2 ↔ tahlo-neco:3
- Mate:377: ruka_zak, deska:1 ↔ tahlo3:4
- Mate:378: ruka_zak, deska:1 ↔ tahlo3:4
- Mate:379: tahlo3:4 ↔ tahlo-neco:3
- Mate:380 (4 mm): clanek3a:1 ↔ ruka_lozisko:1
- Mate:381: tahlo3:4 ↔ packa_prava:1
- Mate:382: tahlo3:4 ↔ packa_prava:1
- Mate:383: ruka_tahlo:4 ↔ packa_prava:1
- Mate:384: kolejnicka_ruka_druha_cast:1 ↔ tahlo6:1
- Mate:385: kolejnicka_ruka_druha_cast:1 ↔ tahlo6:1
- Mate:386: kolejnicka_ruka_druha_cast:1 ↔ tahlo6:1
- Mate:387: tahlo-neco:3 ↔ tahlo6:1
- Mate:388: tahlo-neco:1 ↔ tahlo6:1
- Mate:389: paka2_micro:1 ↔ tahlo5:2
- Mate:390: tahlo6:1 ↔ tahlo5:2
- Mate:391: tahlo6:1 ↔ tahlo5:2
- Mate:392: ruka_zak, deska:1 ↔ paka_packa:1
- Mate:393: ruka_zak, deska:1 ↔ paka_packa:1
- Mate:394: ruka_zak, deska:1 ↔ paka_packa:1
- Mate:395: tahlo3:1 ↔ pracka_leva1:1
